# Autodesk Inventor assembly: EngineAssemblySafe
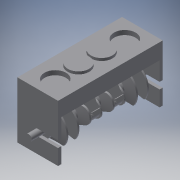
[picture p0: Inventor's stored thumbnail of the model, 180x180]
Saved by Autodesk Inventor 2018 (Build 220112000, 112)
## iProperties
Created: 2019-09-05
Part Number: EngineAssemblySafe
Document SubType Name: Assembly
Designer: 871357
Author: 871357
## Documents named in this file (6)
- L:\Capstone\EngineAssemblySafe.iam
- L:\Capstone\PistonClip.ipt
- L:\Capstone\PistonsHead.ipt
- L:\Capstone\PistonsRod.ipt
- L:\Capstone\Crankshaft.ipt
- L:\Capstone\Engine Block.ipt
## Components (14 placed, 5 different names)
1. PistonClip:1 — Mate:4, Mate:5, Flush:1
2. PistonsHead:1 — Mate:1, Mate:2, Mate:11
3. PistonsRod:1 — Mate:1, Mate:2, Mate:4, Mate:5, Flush:1, Mate:6, Mate:7
4. Crankshaft:1 — Mate:6, Mate:7, Mate:8, Mate:9, Mate:12, Mate:25, Mate:26, Mate:27
5. Engine Block:1 — Mate:8, Mate:9, Mate:11, Mate:12, Mate:28, Mate:29, Mate:30
6. PistonClip:2 — Mate:19, Mate:20, Flush:2
7. PistonClip:3 — Mate:21, Flush:3, Mate:22
8. PistonClip:4 — Mate:23, Flush:4, Mate:24
9. PistonsHead:2 — Mate:13, Mate:14, Mate:28
10. PistonsHead:3 — Mate:15, Mate:16, Mate:29
11. PistonsHead:4 — Mate:17, Mate:18, Mate:30
12. PistonsRod:2 — Mate:13, Mate:14, Mate:19, Mate:20, Flush:2, Mate:25
13. PistonsRod:3 — Mate:15, Mate:16, Mate:21, Flush:3, Mate:22, Mate:26
14. PistonsRod:4 — Mate:17, Mate:18, Mate:23, Flush:4, Mate:24, Mate:27
## Relationships (32: Mate 28, Flush 4)
- Mate:1: PistonsHead:1 ↔ PistonsRod:1
- Mate:2 (-15.875 mm): PistonsHead:1 ↔ PistonsRod:1
- Mate:4 (0.635 mm): PistonClip:1 ↔ PistonsRod:1
- Mate:5 (1.27 mm): PistonClip:1 ↔ PistonsRod:1
- Flush:1: PistonClip:1 ↔ PistonsRod:1
- Mate:6: PistonsRod:1 ↔ Crankshaft:1
- Mate:7 (3.175 mm): PistonsRod:1 ↔ Crankshaft:1
- Mate:8: Crankshaft:1 ↔ Engine Block:1
- Mate:9: Crankshaft:1 ↔ Engine Block:1
- Mate:11: PistonsHead:1 ↔ Engine Block:1
- Mate:12 (7.62 mm): Crankshaft:1 ↔ Engine Block:1
- Mate:13: PistonsHead:2 ↔ PistonsRod:2
- Mate:14 (-15.875 mm): PistonsHead:2 ↔ PistonsRod:2
- Mate:15: PistonsHead:3 ↔ PistonsRod:3
- Mate:16 (-15.875 mm): PistonsHead:3 ↔ PistonsRod:3
- Mate:17: PistonsHead:4 ↔ PistonsRod:4
- Mate:18 (-15.875 mm): PistonsHead:4 ↔ PistonsRod:4
- Mate:19 (0.635 mm): PistonClip:2 ↔ PistonsRod:2
- Mate:20 (0.635 mm): PistonClip:2 ↔ PistonsRod:2
- Flush:2: PistonClip:2 ↔ PistonsRod:2
- Mate:21 (0.635 mm): PistonClip:3 ↔ PistonsRod:3
- Flush:3: PistonClip:3 ↔ PistonsRod:3
- Mate:22 (0.635 mm): PistonClip:3 ↔ PistonsRod:3
- Mate:23 (0.635 mm): PistonClip:4 ↔ PistonsRod:4
- Flush:4: PistonClip:4 ↔ PistonsRod:4
- Mate:24 (0.635 mm): PistonClip:4 ↔ PistonsRod:4
- Mate:25: Crankshaft:1 ↔ PistonsRod:2
- Mate:26: Crankshaft:1 ↔ PistonsRod:3
- Mate:27: Crankshaft:1 ↔ PistonsRod:4
- Mate:28: Engine Block:1 ↔ PistonsHead:2
- Mate:29: Engine Block:1 ↔ PistonsHead:3
- Mate:30: Engine Block:1 ↔ PistonsHead:4
